# Autodesk Inventor assembly: Assembly1
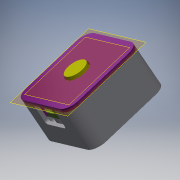
[picture p0: Inventor's stored thumbnail of the model, 180x180]
Saved by Autodesk Inventor 2019 (Build 230136000, 136)
## iProperties
Created: 2019-08-20
Part Number: Assembly1
Document SubType Name: Assembly
Designer: assman
Author: assman
## Documents named in this file (5)
- D:\Inventor\Projects\pushbuttonbox\Assembly1.iam
- D:\Inventor\Projects\pushbuttonbox\board_blueprint.ipt
- D:\Inventor\Projects\pushbuttonbox\bottom.ipt
- D:\Inventor\Projects\pushbuttonbox\button.ipt
- D:\Inventor\Projects\pushbuttonbox\cap.ipt
## Components (4 placed, 4 different names)
1. board_blueprint:1 — Flush:1, Flush:4
2. bottom:1 — Flush:2, Flush:3, Flush:10
3. button:1 — Flush:5, Flush:6, Flush:7, Flush:10
4. cap:1 — Flush:8, Flush:9
## Relationships (10: Flush 10)
- Flush:1 (1 mm): board_blueprint:1
- Flush:2: bottom:1
- Flush:3: bottom:1
- Flush:4 (0.5 mm): board_blueprint:1
- Flush:5: button:1
- Flush:6: button:1
- Flush:7 (0.2 mm): button:1
- Flush:8: cap:1
- Flush:9: cap:1
- Flush:10: bottom:1 ↔ button:1
